# Autodesk Inventor assembly: robot rev 2
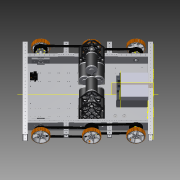
[picture p0: Inventor's stored thumbnail of the model, 180x180]
Saved by Autodesk Inventor 2014 (Build 180170000, 170)
## iProperties
Created: 2014-01-05
Part Number: robot rev 2
Document SubType Name: Assembly
Designer: Arpan
Mass: 55221.5 g
Surface Area: 119399 cm^2
Volume: 30372.2 cm^3
Density: 1.81816 g/cm^3
Author: Arpan
## Documents named in this file (12)
- C:\Users\intern\Documents\GitHub\2014buildCAD\robot rev 2.iam
- C:\Users\intern\Documents\GitHub\2014buildCAD\chassisdrivetrain\chassis light\chassisstructure.iam
- C:\Users\intern\Documents\GitHub\2014buildCAD\electrical\CS_compactRIO_cRIO-FRC-II.ipt
- C:\Users\intern\Documents\GitHub\2014buildCAD\electrical\Pneumatic_Compressor_VIAIR_00090\Pneumatic_Compressor_VIAIR_00090.iam
- C:\Users\intern\Documents\GitHub\2014buildCAD\electrical\CS_PowerBoard_A003206.ipt
- C:\Users\intern\Documents\GitHub\2014buildCAD\electrical\New folder\Talon with Fan.iam
- C:\Users\intern\Documents\GitHub\2014buildCAD\electrical\battery\ELEC_Battery_NP18-12B.iam
- C:\Users\intern\Documents\GitHub\2014buildCAD\shooter arpan\mcmaster carr 32 tooth timing belt.ipt
- C:\Users\intern\Documents\GitHub\2014buildCAD\electrical\CS_Relay_SPIKE-RELAY-H.ipt
- C:\Users\intern\Documents\GitHub\2014buildCAD\chassisdrivetrain\brandons encoders\MagnetHolder 6mm.ipt
- C:\Users\intern\Documents\GitHub\2014buildCAD\chassisdrivetrain\brandons encoders\Magnet.ipt
- C:\Users\intern\Documents\GitHub\2014buildCAD\chassisdrivetrain\brandons encoders\boardHolderv2.ipt
## Components (23 placed, 11 different names)
1. chassisstructure:1 [sub-assembly] — Mate:1, Mate:2, Mate:4, Mate:5, Mate:6, Mate:7, Mate:8, Mate:9, Mate:10, Mate:11, Mate:12, Mate:15, Mate:16, Mate:17, Mate:18, Mate:25, Mate:26, Mate:29, Mate:30, Mate:31, Mate:41, Flush:14, Mate:47, Mate:48, Mate:49, Mate:51, Mate:52, Mate:53, Mate:54, Mate:57, Mate:58, Mate:59, Mate:62, Angle:1
2. CS_compactRIO_cRIO-FRC-II:1 — Mate:1, Mate:25, Mate:26
3. Pneumatic_Compressor_VIAIR_00090:1 [sub-assembly] — Mate:2, Mate:29, Mate:30, Mate:31
4. CS_PowerBoard_A003206:1 — Mate:4, Mate:15, Mate:23, Mate:24, Mate:41
5. Talon with Fan:1 [sub-assembly] — Mate:12, Flush:3, Flush:9, Flush:10, Mate:19
6. Talon with Fan:2 [sub-assembly] — Mate:11, Flush:1, Flush:2, Flush:3, Flush:6, Mate:22
7. Talon with Fan:3 [sub-assembly] — Mate:9, Flush:1, Flush:7, Mate:22
8. Talon with Fan:4 [sub-assembly] — Mate:10, Flush:2, Flush:8, Mate:24
9. Talon with Fan:5 [sub-assembly] — Mate:6, Mate:13, Flush:5, Flush:6
10. Talon with Fan:6 [sub-assembly] — Mate:5, Flush:4, Flush:8, Mate:20, Mate:21
11. Talon with Fan:7 [sub-assembly] — Mate:8, Mate:13, Flush:4, Flush:7, Mate:21
12. Talon with Fan:8 [sub-assembly] — Mate:7, Flush:5, Flush:9, Flush:11, Mate:20, Mate:23
13. Talon with Fan:9 [sub-assembly] — Mate:16, Flush:11, Flush:12, Mate:50
14. Talon with Fan:10 [sub-assembly] — Mate:17, Flush:10, Flush:12, Mate:18, Mate:19
15. ELEC_Battery_NP18-12B:1 [sub-assembly] — Mate:47
16. mcmaster carr 32 tooth timing belt:1
17. CS_Relay_SPIKE-RELAY-H:1 — Mate:48, Mate:49, Mate:50
18. MagnetHolder 6mm:1 — Insert:1, Mate:51, Mate:52, Mate:53
19. Magnet:1 — Insert:1, Mate:55
20. boardHolderv2:1 — Mate:54, Mate:56
21. boardHolderv2:2 — Mate:61, Mate:62, Angle:1
22. MagnetHolder 6mm:2 — Mate:57, Mate:58, Mate:59, Insert:2
23. Magnet:2 — Insert:2, Mate:60
## Relationships (60: Mate 44, Flush 13, Insert 2, Angle 1)
- Mate:1: chassisstructure:1 ↔ CS_compactRIO_cRIO-FRC-II:1
- Mate:2: chassisstructure:1 ↔ Pneumatic_Compressor_VIAIR_00090:1
- Mate:4: chassisstructure:1 ↔ CS_PowerBoard_A003206:1
- Mate:5: chassisstructure:1 ↔ Talon with Fan:6
- Mate:6: chassisstructure:1 ↔ Talon with Fan:5
- Mate:7: chassisstructure:1 ↔ Talon with Fan:8
- Mate:8: chassisstructure:1 ↔ Talon with Fan:7
- Mate:9: chassisstructure:1 ↔ Talon with Fan:3
- Mate:10: chassisstructure:1 ↔ Talon with Fan:4
- Mate:11: chassisstructure:1 ↔ Talon with Fan:2
- Mate:12: chassisstructure:1 ↔ Talon with Fan:1
- Flush:1: Talon with Fan:2 ↔ Talon with Fan:3
- Flush:2: Talon with Fan:2 ↔ Talon with Fan:4
- Flush:3: Talon with Fan:1 ↔ Talon with Fan:2
- Mate:13: Talon with Fan:5 ↔ Talon with Fan:7
- Flush:4: Talon with Fan:6 ↔ Talon with Fan:7
- Flush:5: Talon with Fan:5 ↔ Talon with Fan:8
- Flush:6: Talon with Fan:2 ↔ Talon with Fan:5
- Flush:7: Talon with Fan:3 ↔ Talon with Fan:7
- Flush:8: Talon with Fan:4 ↔ Talon with Fan:6
- Flush:9: Talon with Fan:1 ↔ Talon with Fan:8
- Mate:15 (161.2646 mm): chassisstructure:1 ↔ CS_PowerBoard_A003206:1
- Mate:16: chassisstructure:1 ↔ Talon with Fan:9
- Mate:17: chassisstructure:1 ↔ Talon with Fan:10
- Flush:10: Talon with Fan:1 ↔ Talon with Fan:10
- Flush:11: Talon with Fan:8 ↔ Talon with Fan:9
- Flush:12: Talon with Fan:9 ↔ Talon with Fan:10
- Mate:18 (12.7 mm): chassisstructure:1 ↔ Talon with Fan:10
- Mate:19 (3.175 mm): Talon with Fan:1 ↔ Talon with Fan:10
- Mate:20 (3.175 mm): Talon with Fan:6 ↔ Talon with Fan:8
- Mate:21 (3.175 mm): Talon with Fan:6 ↔ Talon with Fan:7
- Mate:22 (3.175 mm): Talon with Fan:2 ↔ Talon with Fan:3
- Mate:23 (25.4 mm): CS_PowerBoard_A003206:1 ↔ Talon with Fan:8
- Mate:24 (25.4 mm): CS_PowerBoard_A003206:1 ↔ Talon with Fan:4
- Mate:25 (25.4 mm): chassisstructure:1 ↔ CS_compactRIO_cRIO-FRC-II:1
- Mate:26 (25.4 mm): chassisstructure:1 ↔ CS_compactRIO_cRIO-FRC-II:1
- Mate:29 (25.4 mm): chassisstructure:1 ↔ Pneumatic_Compressor_VIAIR_00090:1
- Mate:30 (25.4 mm): chassisstructure:1 ↔ Pneumatic_Compressor_VIAIR_00090:1
- Mate:31 (25.4 mm): chassisstructure:1 ↔ Pneumatic_Compressor_VIAIR_00090:1
- Mate:41: chassisstructure:1 ↔ CS_PowerBoard_A003206:1
- Flush:14 (25.4 mm): chassisstructure:1
- Mate:47: chassisstructure:1 ↔ ELEC_Battery_NP18-12B:1
- Mate:48: chassisstructure:1 ↔ CS_Relay_SPIKE-RELAY-H:1
- Mate:49 (12.7 mm): chassisstructure:1 ↔ CS_Relay_SPIKE-RELAY-H:1
- Mate:50 (11.5062 mm): Talon with Fan:9 ↔ CS_Relay_SPIKE-RELAY-H:1
- Insert:1: MagnetHolder 6mm:1 ↔ Magnet:1
- Mate:51: chassisstructure:1 ↔ MagnetHolder 6mm:1
- Mate:52: chassisstructure:1 ↔ MagnetHolder 6mm:1
- Mate:53: chassisstructure:1 ↔ MagnetHolder 6mm:1
- Mate:54: chassisstructure:1 ↔ boardHolderv2:1
- Mate:55: Magnet:1
- Mate:56: boardHolderv2:1
- Mate:57: chassisstructure:1 ↔ MagnetHolder 6mm:2
- Mate:58: chassisstructure:1 ↔ MagnetHolder 6mm:2
- Mate:59: chassisstructure:1 ↔ MagnetHolder 6mm:2
- Insert:2: MagnetHolder 6mm:2 ↔ Magnet:2
- Mate:60: Magnet:2
- Mate:61: boardHolderv2:2
- Mate:62: chassisstructure:1 ↔ boardHolderv2:2
- Angle:1 (0 deg): chassisstructure:1 ↔ boardHolderv2:2
